# Autodesk Inventor assembly: Boat_Bot_Assembly
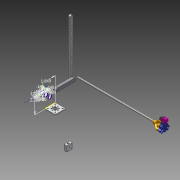
[picture p0: Inventor's stored thumbnail of the model, 180x180]
Saved by Autodesk Inventor 2014 SP1 (Build 180222100, 222)
## iProperties
Created: 2014-01-22
Part Number: Boat_Bot_Assembly
Document SubType Name: Assembly
Designer: tom
Author: tom
## Documents named in this file (10)
- C:\Users\tom\Documents\GitHub\Boat_Bot\Boat_Bot_Assembly.iam
- C:\Users\tom\Documents\GitHub\Belt_Cutter\Beam2.ipt
- C:\Users\tom\Documents\GitHub\Boat_Bot\Arm Tube.ipt
- C:\Users\tom\Documents\GitHub\Boat_Bot\Base.ipt
- C:\Users\tom\Documents\GitHub\Boat_Bot\Channel Bracket B.ipt
- C:\Users\tom\Documents\GitHub\Boat_Bot\Tube Bracket.ipt
- C:\Users\tom\Documents\GitHub\Boat_Bot\Coupler.ipt
- C:\Users\tom\Documents\GitHub\Boat_Bot\Plunger2.ipt
- C:\Users\tom\Documents\GitHub\Boat_Bot\Finger Joint.ipt
- C:\Users\tom\Documents\GitHub\Boat_Bot\linkage.ipt
## Components (9 placed, 9 different names)
1. Base:1 — Mate:1, Rotational:1
2. Arm Tube:1 — Mate:2
3. Beam2:1 — Rotational:1
4. Channel Bracket B:1
5. Tube Bracket:1
6. Coupler:1 — Mate:2, Rotational:2
7. Plunger2:1 — Rotational:3
8. Finger:1 — Rotational:3
9. linkage:1 — Rotational:2
## Relationships (5: RevoluteJoint 3, Mate 2)
- Mate:1: Base:1
- Rotational:1 [RevoluteJoint]: Base:1 ↔ Beam2:1
- Mate:2: Arm Tube:1 ↔ Coupler:1
- Rotational:2 [RevoluteJoint]: Coupler:1 ↔ linkage:1
- Rotational:3 [RevoluteJoint]: Plunger2:1 ↔ Finger:1
